# Autodesk Inventor assembly: 5 Barras Simplificado
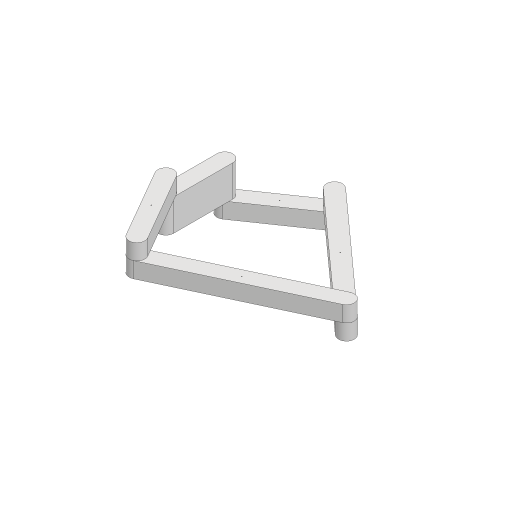
[picture p0: Inventor's stored thumbnail of the model, 512x512]
Saved by Autodesk Inventor 2024.2 (Build 282272000, 272)
## iProperties
Created: 2025-02-22
Part Number: 5 Barras Simplificado
Document SubType Name: Assembly
Designer: jp.reyesf
Author: jp.reyesf
## Documents named in this file (6)
- C:\Users\jp.reyesf\Desktop\Master-Thesis\five_bar\assets\CAD\5 Barras Simplificado.iam
- C:\Users\jp.reyesf\Desktop\Master-Thesis\five_bar\assets\CAD\Solid6.ipt
- C:\Users\jp.reyesf\Desktop\Master-Thesis\five_bar\assets\CAD\Solid7.ipt
- C:\Users\jp.reyesf\Desktop\Master-Thesis\five_bar\assets\CAD\Solid8.ipt
- C:\Users\jp.reyesf\Desktop\Master-Thesis\five_bar\assets\CAD\Solid9.ipt
- C:\Users\jp.reyesf\Desktop\Master-Thesis\five_bar\assets\CAD\Solid10.ipt
## Components (5 placed, 5 different names)
1. Solid6:1 — Mate:1, Mate:2, Mate:6, Mate:7
2. Solid7:1 — Mate:2, Mate:3, Mate:7, Mate:10
3. Solid8:1 — Mate:3, Mate:4, Mate:10
4. Solid9:1 — Mate:4, Mate:5, Mate:9
5. Solid10:1 — Mate:1, Mate:5, Mate:6, Mate:9
## Relationships (9: Mate 9)
- Mate:1: Solid6:1 ↔ Solid10:1
- Mate:2: Solid6:1 ↔ Solid7:1
- Mate:3: Solid7:1 ↔ Solid8:1
- Mate:4: Solid8:1 ↔ Solid9:1
- Mate:5: Solid9:1 ↔ Solid10:1
- Mate:6: Solid6:1 ↔ Solid10:1
- Mate:7: Solid6:1 ↔ Solid7:1
- Mate:9: Solid9:1 ↔ Solid10:1
- Mate:10: Solid7:1 ↔ Solid8:1
